# Autodesk Inventor assembly: ASY Beshkino main
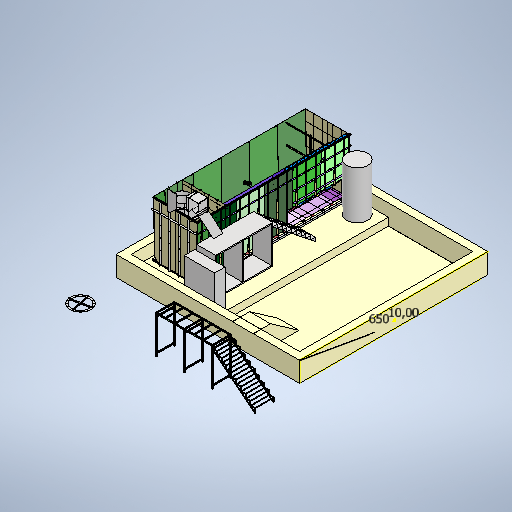
[picture p0: Inventor's stored thumbnail of the model, 512x512]
Saved by Autodesk Inventor 2025 (Build 290162010, 162A)
## iProperties
Created: 2024-08-27
Part Number: ASY Beshkino main
Document SubType Name: Assembly
Designer: DELL
Author: DELL
## Documents named in this file (12)
- C:\Users\admin\YandexDisk-badmisterfox\домашниий пк\Inventor\BSH_Beshkino_bio_tank\ASY Beshkino main.iam
- C:\Users\admin\YandexDisk-badmisterfox\домашниий пк\Inventor\BSH_Beshkino_bio_tank\BSH 0 foudation.ipt
- C:\Users\admin\YandexDisk-badmisterfox\домашниий пк\Inventor\BSH_Beshkino_bio_tank\ASY Beshkino_bio_tank.iam
- C:\Users\admin\YandexDisk-badmisterfox\домашниий пк\Inventor\BSH_Beshkino_bio_tank\ASY Trommel.iam
- C:\Users\admin\YandexDisk-badmisterfox\домашниий пк\Inventor\BSH_Beshkino_bio_tank\3d party\RXm3 assieme dimensionale mag2018.ipt
- C:\Users\admin\YandexDisk-badmisterfox\домашниий пк\Inventor\BSH_Beshkino_bio_tank\3d party\motor-reductor NMRV040\motor-reductor NMRV040.iam
- C:\Users\admin\YandexDisk-badmisterfox\домашниий пк\Inventor\BSH_Beshkino_bio_tank\BSH 01 foam filter.ipt
- C:\Users\admin\YandexDisk-badmisterfox\домашниий пк\Inventor\BSH_Beshkino_bio_tank\BSH 01 bag.ipt
- C:\Users\admin\YandexDisk-badmisterfox\домашниий пк\Inventor\BSH_Beshkino_bio_tank\BSH 03 upstairs.ipt
- C:\Users\admin\YandexDisk-badmisterfox\домашниий пк\Inventor\BSH_Beshkino_bio_tank\лестница\Перегородка\ASY NDM 11.0 перегородка.iam
- C:\Users\admin\YandexDisk-badmisterfox\домашниий пк\Inventor\BSH_Beshkino_bio_tank\Конструкция.iam
- C:\Users\admin\YandexDisk-badmisterfox\домашниий пк\Inventor\BSH_Beshkino_bio_tank\ASY BSH 500 cap.iam
## Components (12 placed, 11 different names)
1. BSH 0 foudation:1 — Mate:1, Mate:2, Mate:3, Mate:4, Flush:2, Flush:3, Flush:4
2. ASY Beshkino_bio_tank:1 [sub-assembly] — Mate:2, Mate:3, Mate:4, Flush:1, Mate:5, Mate:6
3. ASY Trommel:1 [sub-assembly] — Flush:1
4. RXm3 assieme dimensionale mag2018:1 — Mate:5
5. RXm3 assieme dimensionale mag2018:2 — Mate:6
6. motor-reductor NMRV040:1 [sub-assembly]
7. BSH 01 foam filter:1 — Flush:2
8. BSH 01 bag:1 — Flush:3
9. BSH 03 upstairs:1 — Flush:4
10. ASY NDM 11.0 перегородка:1 [sub-assembly]
11. Конструкция:1 [sub-assembly]
12. ASY BSH 500 cap:1 [sub-assembly]
## Relationships (10: Mate 6, Flush 4)
- Mate:1: BSH 0 foudation:1
- Mate:2: BSH 0 foudation:1 ↔ ASY Beshkino_bio_tank:1
- Mate:3 (100 mm): BSH 0 foudation:1 ↔ ASY Beshkino_bio_tank:1
- Mate:4 (200 mm): BSH 0 foudation:1 ↔ ASY Beshkino_bio_tank:1
- Flush:1: ASY Beshkino_bio_tank:1 ↔ ASY Trommel:1
- Mate:5: ASY Beshkino_bio_tank:1 ↔ RXm3 assieme dimensionale mag2018:1
- Mate:6: ASY Beshkino_bio_tank:1 ↔ RXm3 assieme dimensionale mag2018:2
- Flush:2: BSH 0 foudation:1 ↔ BSH 01 foam filter:1
- Flush:3: BSH 0 foudation:1 ↔ BSH 01 bag:1
- Flush:4: BSH 0 foudation:1 ↔ BSH 03 upstairs:1
